# Autodesk Inventor assembly: ConveyorFrame
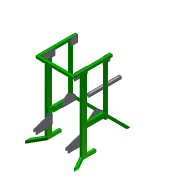
[picture p0: Inventor's stored thumbnail of the model, 180x180]
Saved by Autodesk Inventor 2012 (Build 160160000, 160)
## iProperties
Created: 2012-01-09
Part Number: ConveyorFrame
Document SubType Name: Assembly
Designer: JesseK
Mass: 4568.77 g
Surface Area: 14901.2 cm^2
Volume: 1926.67 cm^3
Density: 2.37132 g/cm^3
Author: JesseK
## Documents named in this file (14)
- Z:\UserData\Documents\Inventor\team1885frc\Robot2012\Conveyor\ConveyorFrame.iam
- Z:\UserData\Documents\Inventor\team1885frc\Robot2012\Conveyor\Conveyor_Frame_FrontTallRail_2x1.ipt
- Z:\UserData\Documents\Inventor\team1885frc\Robot2012\Conveyor\Frame_ConveyorMountRail.ipt
- Z:\UserData\Documents\Inventor\team1885frc\Robot2012\Conveyor\Frame_FrontAngle.ipt
- Z:\UserData\Documents\Inventor\team1885frc\Robot2012\Conveyor\Frame_TopRail.ipt
- Z:\UserData\Documents\Inventor\team1885frc\Robot2012\Conveyor\Frame_TopCrossRail.ipt
- Z:\UserData\Documents\Inventor\team1885frc\Robot2012\Conveyor\Frame_BottomRollerPlate.ipt
- Z:\UserData\Documents\Inventor\team1885frc\Robot2012\Conveyor\Frame_TopFrontRollerPlate.ipt
- Z:\UserData\Documents\Inventor\team1885frc\Robot2012\Conveyor\Frame_MidRollerSupport.ipt
- Z:\UserData\Documents\Inventor\team1885frc\Robot2012\Conveyor\Frame_MidRollerPlate.ipt
- Z:\UserData\Documents\Inventor\team1885frc\Robot2012\Conveyor\Frame_RearLowerAngleSupport.ipt
- Z:\UserData\Documents\Inventor\team1885frc\Robot2012\Conveyor\Frame_RearVerticalSupport.ipt
- Z:\UserData\Documents\Inventor\team1885frc\Robot2012\Conveyor\Frame_TopRearRollerPlate.ipt
- Z:\UserData\Documents\Inventor\team1885frc\Robot2012\Conveyor\Frame_RearBallGuideSupport.ipt
## Components (24 placed, 13 different names)
1. Conveyor_Frame_FrontTallRail_2x1:1 — Mate:6, Flush:4, Flush:5, Mate:7, Mate:9, Flush:7, Mate:10, Mate:15, Mate:16, Mate:18, Mate:22, Mate:23, Mate:24, Mate:26, Mate:39, Mate:40
2. Conveyor_Frame_FrontTallRail_2x1:2 — Flush:3, Mate:5, Flush:5, Mate:7, Flush:8, Mate:11, Mate:14, Flush:12, Mate:17, Mate:19, Mate:20, Mate:21, Mate:25, Mate:37, Mate:38
3. Frame_ConveyorMountRail:1 — Flush:1, Mate:1, Mate:2, Flush:3, Mate:5, Mate:8, Mate:45
4. Frame_FrontAngle:1 — Flush:1, Mate:1, Mate:2, Flush:6
5. Frame_ConveyorMountRail:2 — Flush:2, Mate:3, Mate:4, Mate:6, Flush:4, Mate:8, Mate:42
6. Frame_FrontAngle:2 — Flush:2, Mate:3, Mate:4, Flush:6, Mate:9
7. Frame_TopRail:1 — Flush:8, Mate:11, Mate:12, Flush:9, Mate:57, Mate:58, Mate:59
8. Frame_TopRail:2 — Flush:7, Mate:10, Mate:12, Flush:10, Mate:13, Mate:53, Mate:54, Mate:55
9. Frame_TopCrossRail:1 — Flush:9, Flush:10, Mate:13
10. Frame_BottomRollerPlate:1 — Mate:14, Flush:11, Flush:12, Mate:17
11. Frame_BottomRollerPlate:2 — Mate:15, Flush:11, Mate:16, Mate:18
12. Frame_TopFrontRollerPlate:1 — Mate:22, Mate:23, Mate:24
13. Frame_TopFrontRollerPlate:2 — Mate:19, Mate:20, Mate:21
14. Frame_MidRollerSupport:1 — Mate:26, Mate:31, Mate:35, Mate:36, Mate:39, Mate:40, Mate:41, Mate:43, Mate:47, Mate:48, Mate:49
15. Frame_MidRollerSupport:2 — Mate:25, Mate:32, Mate:33, Mate:34, Mate:37, Mate:38, Mate:44, Mate:46, Mate:50, Mate:51, Mate:52
16. Frame_MidRollerPlate:1 — Mate:32, Mate:33, Mate:34
17. Frame_MidRollerPlate:2 — Mate:31, Mate:35, Mate:36
18. Frame_RearLowerAngleSupport:1 — Mate:44, Mate:45, Mate:46
19. Frame_RearLowerAngleSupport:2 — Mate:41, Mate:42, Mate:43
20. Frame_RearVerticalSupport:1 — Mate:50, Mate:51, Mate:52
21. Frame_RearVerticalSupport:2 — Mate:47, Mate:48, Mate:49, Mate:56
22. Frame_TopRearRollerPlate:1 — Mate:53, Mate:54, Mate:55, Mate:56
23. Frame_TopRearRollerPlate:2 — Mate:57, Mate:58, Mate:59
24. Frame_RearBallGuideSupport:1
## Relationships (67: Mate 55, Flush 12)
- Flush:1: Frame_ConveyorMountRail:1 ↔ Frame_FrontAngle:1
- Mate:1: Frame_ConveyorMountRail:1 ↔ Frame_FrontAngle:1
- Mate:2: Frame_ConveyorMountRail:1 ↔ Frame_FrontAngle:1
- Flush:2: Frame_ConveyorMountRail:2 ↔ Frame_FrontAngle:2
- Mate:3: Frame_ConveyorMountRail:2 ↔ Frame_FrontAngle:2
- Mate:4: Frame_ConveyorMountRail:2 ↔ Frame_FrontAngle:2
- Flush:3: Conveyor_Frame_FrontTallRail_2x1:2 ↔ Frame_ConveyorMountRail:1
- Mate:5: Conveyor_Frame_FrontTallRail_2x1:2 ↔ Frame_ConveyorMountRail:1
- Mate:6: Conveyor_Frame_FrontTallRail_2x1:1 ↔ Frame_ConveyorMountRail:2
- Flush:4: Conveyor_Frame_FrontTallRail_2x1:1 ↔ Frame_ConveyorMountRail:2
- Flush:5: Conveyor_Frame_FrontTallRail_2x1:1 ↔ Conveyor_Frame_FrontTallRail_2x1:2
- Mate:7 (355.6 mm): Conveyor_Frame_FrontTallRail_2x1:1 ↔ Conveyor_Frame_FrontTallRail_2x1:2
- Flush:6: Frame_FrontAngle:1 ↔ Frame_FrontAngle:2
- Mate:8: Frame_ConveyorMountRail:1 ↔ Frame_ConveyorMountRail:2
- Mate:9 (152.4 mm): Conveyor_Frame_FrontTallRail_2x1:1 ↔ Frame_FrontAngle:2
- Flush:7: Conveyor_Frame_FrontTallRail_2x1:1 ↔ Frame_TopRail:2
- Mate:10: Conveyor_Frame_FrontTallRail_2x1:1 ↔ Frame_TopRail:2
- Flush:8: Conveyor_Frame_FrontTallRail_2x1:2 ↔ Frame_TopRail:1
- Mate:11: Conveyor_Frame_FrontTallRail_2x1:2 ↔ Frame_TopRail:1
- Mate:12: Frame_TopRail:1 ↔ Frame_TopRail:2
- Flush:9: Frame_TopRail:1 ↔ Frame_TopCrossRail:1
- Flush:10: Frame_TopRail:2 ↔ Frame_TopCrossRail:1
- Mate:13: Frame_TopRail:2 ↔ Frame_TopCrossRail:1
- Mate:14: Conveyor_Frame_FrontTallRail_2x1:2 ↔ Frame_BottomRollerPlate:1
- Mate:15: Conveyor_Frame_FrontTallRail_2x1:1 ↔ Frame_BottomRollerPlate:2
- Flush:11: Frame_BottomRollerPlate:1 ↔ Frame_BottomRollerPlate:2
- Flush:12: Conveyor_Frame_FrontTallRail_2x1:2 ↔ Frame_BottomRollerPlate:1
- Mate:16: Conveyor_Frame_FrontTallRail_2x1:1 ↔ Frame_BottomRollerPlate:2
- Mate:17: Conveyor_Frame_FrontTallRail_2x1:2 ↔ Frame_BottomRollerPlate:1
- Mate:18: Conveyor_Frame_FrontTallRail_2x1:1 ↔ Frame_BottomRollerPlate:2
- Mate:19: Conveyor_Frame_FrontTallRail_2x1:2 ↔ Frame_TopFrontRollerPlate:2
- Mate:20: Conveyor_Frame_FrontTallRail_2x1:2 ↔ Frame_TopFrontRollerPlate:2
- Mate:21: Conveyor_Frame_FrontTallRail_2x1:2 ↔ Frame_TopFrontRollerPlate:2
- Mate:22: Conveyor_Frame_FrontTallRail_2x1:1 ↔ Frame_TopFrontRollerPlate:1
- Mate:23: Conveyor_Frame_FrontTallRail_2x1:1 ↔ Frame_TopFrontRollerPlate:1
- Mate:24: Conveyor_Frame_FrontTallRail_2x1:1 ↔ Frame_TopFrontRollerPlate:1
- Mate:25: Conveyor_Frame_FrontTallRail_2x1:2 ↔ Frame_MidRollerSupport:2
- Mate:26: Conveyor_Frame_FrontTallRail_2x1:1 ↔ Frame_MidRollerSupport:1
- Mate:31: Frame_MidRollerSupport:1 ↔ Frame_MidRollerPlate:2
- Mate:32: Frame_MidRollerSupport:2 ↔ Frame_MidRollerPlate:1
- Mate:33: Frame_MidRollerSupport:2 ↔ Frame_MidRollerPlate:1
- Mate:34: Frame_MidRollerSupport:2 ↔ Frame_MidRollerPlate:1
- Mate:35: Frame_MidRollerSupport:1 ↔ Frame_MidRollerPlate:2
- Mate:36: Frame_MidRollerSupport:1 ↔ Frame_MidRollerPlate:2
- Mate:37: Conveyor_Frame_FrontTallRail_2x1:2 ↔ Frame_MidRollerSupport:2
- Mate:38: Conveyor_Frame_FrontTallRail_2x1:2 ↔ Frame_MidRollerSupport:2
- Mate:39: Conveyor_Frame_FrontTallRail_2x1:1 ↔ Frame_MidRollerSupport:1
- Mate:40: Conveyor_Frame_FrontTallRail_2x1:1 ↔ Frame_MidRollerSupport:1
- Mate:41: Frame_MidRollerSupport:1 ↔ Frame_RearLowerAngleSupport:2
- Mate:42: Frame_ConveyorMountRail:2 ↔ Frame_RearLowerAngleSupport:2
- Mate:43: Frame_MidRollerSupport:1 ↔ Frame_RearLowerAngleSupport:2
- Mate:44: Frame_MidRollerSupport:2 ↔ Frame_RearLowerAngleSupport:1
- Mate:45: Frame_ConveyorMountRail:1 ↔ Frame_RearLowerAngleSupport:1
- Mate:46: Frame_MidRollerSupport:2 ↔ Frame_RearLowerAngleSupport:1
- Mate:47: Frame_MidRollerSupport:1 ↔ Frame_RearVerticalSupport:2
- Mate:48: Frame_MidRollerSupport:1 ↔ Frame_RearVerticalSupport:2
- Mate:49: Frame_MidRollerSupport:1 ↔ Frame_RearVerticalSupport:2
- Mate:50: Frame_MidRollerSupport:2 ↔ Frame_RearVerticalSupport:1
- Mate:51: Frame_MidRollerSupport:2 ↔ Frame_RearVerticalSupport:1
- Mate:52: Frame_MidRollerSupport:2 ↔ Frame_RearVerticalSupport:1
- Mate:53: Frame_TopRail:2 ↔ Frame_TopRearRollerPlate:1
- Mate:54: Frame_TopRail:2 ↔ Frame_TopRearRollerPlate:1
- Mate:55: Frame_TopRail:2 ↔ Frame_TopRearRollerPlate:1
- Mate:56: Frame_RearVerticalSupport:2 ↔ Frame_TopRearRollerPlate:1
- Mate:57: Frame_TopRail:1 ↔ Frame_TopRearRollerPlate:2
- Mate:58: Frame_TopRail:1 ↔ Frame_TopRearRollerPlate:2
- Mate:59: Frame_TopRail:1 ↔ Frame_TopRearRollerPlate:2
